# Autodesk Inventor assembly: ASY МОО 001 отстойник осветлитель
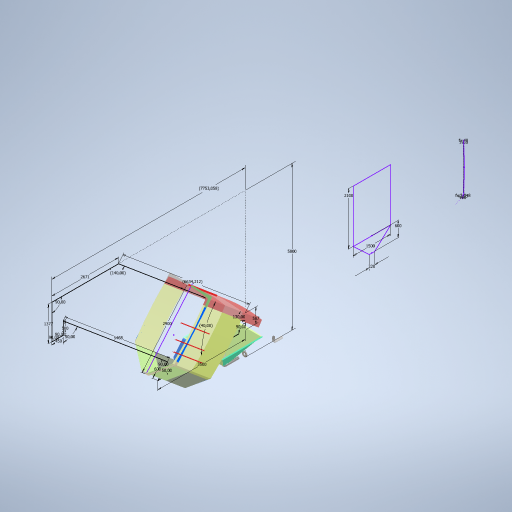
[picture p0: Inventor's stored thumbnail of the model, 512x512]
Saved by Autodesk Inventor 2024.2 (Build 282272000, 272)
## iProperties
Created: 2024-04-28
Part Number: ASY МОО 001 отстойник осветлитель
Document SubType Name: Weldment
Designer: admin
Weld Material: Welded Aluminum-6061
Mass: 420020 g
Surface Area: 719213 cm^2
Volume: 106788 cm^3
Density: 3.93322 g/cm^3
Author: admin
## Documents named in this file (23)
- C:\Users\user\YandexDisk\домашниий пк\Inventor\Manturovo\Manturovo_Se-clar\ASY МОО 001 отстойник осветлитель.iam
- C:\Users\user\YandexDisk\домашниий пк\Inventor\Manturovo\Manturovo_Se-clar\МОО 020 лист борт 1.ipt
- C:\Users\user\YandexDisk\домашниий пк\Inventor\Manturovo\Manturovo_Se-clar\МОО 010 лист спина 1.ipt
- C:\Users\user\YandexDisk\домашниий пк\Inventor\Manturovo\Manturovo_Se-clar\Пример емкости.ipt
- C:\Users\user\YandexDisk\домашниий пк\Inventor\Manturovo\Manturovo_Se-clar\МОО 030 лист брюхо 1.ipt
- C:\Users\user\YandexDisk\домашниий пк\Inventor\Manturovo\Manturovo_Se-clar\МОО 040 шпангоут борт 1.ipt
- C:\Users\user\YandexDisk\домашниий пк\Inventor\Manturovo\Manturovo_Se-clar\МОО 041 шпангоут спина 1.ipt
- C:\Users\user\YandexDisk\домашниий пк\Inventor\Manturovo\Manturovo_Se-clar\МОО 050 стрингер спина 1.ipt
- C:\Users\user\YandexDisk\домашниий пк\Inventor\Manturovo\Manturovo_Se-clar\Рама основания\ASY МОО 040 рама основания.iam
- C:\Users\user\YandexDisk\домашниий пк\Inventor\Manturovo\Manturovo_Se-clar\ASY МОО 060 ракета.iam
- C:\Users\user\YandexDisk\домашниий пк\Inventor\Manturovo\Manturovo_Se-clar\Content Center Files\en-US\ISO 5251 B 3D\ISO 5251 Bends 3D without straight ends(90 deg) DN80 2 2.ipt
- C:\Users\user\YandexDisk\домашниий пк\Inventor\Manturovo\Manturovo_Se-clar\Content Center Files\en-US\ISO 5251(1)\ISO 5251 Concentric reducers DN80 x DN65 3,2 3,2.ipt
- C:\Users\user\YandexDisk\домашниий пк\Inventor\Manturovo\Manturovo_Se-clar\ASY МОО 020 конус.iam
- C:\Users\user\YandexDisk\домашниий пк\Inventor\Manturovo\Manturovo_Se-clar\ракета\МОО 064 ракета труба.ipt
- C:\Users\user\YandexDisk\домашниий пк\Inventor\Manturovo\Manturovo_Se-clar\х_размеры МОО отстойник осветлитель Dummu.ipt
- C:\Users\user\YandexDisk\домашниий пк\Inventor\Manturovo\Manturovo_Se-clar\МОО 012 лист спина 2.ipt
- C:\Users\user\YandexDisk\домашниий пк\Inventor\Manturovo\Manturovo_Se-clar\ракета\МОО 065 ракета труба 5.ipt
- C:\Users\user\YandexDisk\домашниий пк\Inventor\Manturovo\Manturovo_Se-clar\ракета\МОО 066 ракета труба 6.ipt
- C:\Users\user\YandexDisk\домашниий пк\Inventor\Manturovo\Manturovo_Se-clar\ракета\МОО 067 ракета труба 7.ipt
- C:\Users\user\YandexDisk\домашниий пк\Inventor\Manturovo\Manturovo_Se-clar\Content Center Files\en-US\DIN EN 1092-1 01 - PN 25\DIN EN 1092-1 Plate Flange for Welding Type 01 - PN 25 80 x 88.9.ipt
- C:\Users\user\YandexDisk\домашниий пк\Inventor\Manturovo\Manturovo_Se-clar\МОО 011 лист борт.ipt
- C:\Users\user\YandexDisk\домашниий пк\Inventor\Manturovo\Manturovo_Se-clar\Листы бака Глеб\МОО 031 Усилитель спина.ipt
- C:\Users\user\YandexDisk\домашниий пк\Inventor\Manturovo\Manturovo_Se-clar\Листы бака Глеб\032 Усилитель левый борт.ipt
## Components (37 placed, 22 different names)
1. Пример емкости:1 — Mate:1, Mate:2, Flush:2
2. х_размеры МОО отстойник осветлитель Dummu:1
3. ASY МОО 040 рама основания:1 [sub-assembly] — Flush:19, Flush:20, Flush:21
4. МОО 020 лист борт 1:2 — Angle:1
5. МОО 010 лист спина 1:1 — Flush:3, Rigid:11, Rigid:12
6. МОО 020 лист борт 1:1 — Rigid:21, Rigid:22
7. МОО 030 лист брюхо 1:1 — Mate:9, Flush:29, Mate:21, Rigid:18
8. МОО 040 шпангоут борт 1:2 — Rigid:20
9. МОО 041 шпангоут спина 1:2 — Flush:12, Flush:33, Tangent:3, Rigid:15, Rigid:19, Flush:37
10. МОО 040 шпангоут борт 1:1 — Rigid:15, Flush:34, Rigid:21, Mate:23, Flush:35, Mate:24, Flush:36
11. МОО 050 стрингер спина 1:2 — Flush:34, Mate:23
12. ASY МОО 060 ракета:1 [sub-assembly] — Flush:23, Rigid:10
13. ISO 5251 Bends 3D without straight ends(90 deg) DN80 2:1 — Rigid:2, Rigid:3
14. ISO 5251 Concentric reducers DN80 x DN65 3,2:1 — Rigid:2, Rigid:10
15. ASY МОО 020 конус:1 [sub-assembly] — Flush:22, Mate:16, Flush:28
16. МОО 064 ракета труба:1 — Rigid:3, Cylindrical:1
17. МОО 010 лист спина 1:2 — Rigid:11, Rigid:13, Flush:31, Tangent:1, Flush:32, Tangent:2, Flush:33, Tangent:3
18. МОО 010 лист спина 1:3 — Flush:24, Rigid:12, Mate:19, Mate:22
19. МОО 012 лист спина 2:1 — Mate:15, Mate:16, Flush:27, Mate:19, Mate:22
20. МОО 065 ракета труба 5:1 — Rigid:5
21. МОО 066 ракета труба 6:1 — Rigid:5, Rigid:6
22. МОО 067 ракета труба 7:1 — Rigid:6, Rigid:7
23. DIN EN 1092-1 Plate Flange for Welding Type 01 - PN 25 80 x 88.9:1 — Flush:25, Flush:26, Mate:18, Cylindrical:1
24. ISO 5251 Concentric reducers DN80 x DN65 3,2:2 — Rigid:7
25. МОО 010 лист спина 1:4 — Rigid:13
26. МОО 011 лист борт:1 — Flush:30, Flush:31, Tangent:1, Rigid:16
27. МОО 011 лист борт:2 — Flush:29, Mate:20, Flush:32, Tangent:2, Mate:21
28. МОО 031 Усилитель спина:1
29. 032 Усилитель левый борт:1
30. МОО 041 шпангоут спина 1:3 — Rigid:19, Rigid:20
31. МОО 011 лист борт:3 — Rigid:16, Rigid:17
32. МОО 011 лист борт:4 — Rigid:17
33. МОО 030 лист брюхо 1:2 — Rigid:18
34. МОО 020 лист борт 1:3 — Rigid:22
35. МОО 050 стрингер спина 1:3 — Flush:35, Mate:24
36. МОО 050 стрингер спина 1:4 — Flush:36
37. МОО 050 стрингер спина 1:5 — Flush:37
## Relationships (56: Flush 22, WeldJoint 17, Mate 12, Tangent 3, Angle 1, CylindricalJoint 1)
- Mate:1: Пример емкости:1
- Mate:2: Пример емкости:1
- Flush:2: Пример емкости:1
- Flush:3: МОО 010 лист спина 1:1
- Angle:1 (180 deg): МОО 020 лист борт 1:2
- Mate:9: МОО 030 лист брюхо 1:1
- Flush:12: МОО 041 шпангоут спина 1:2
- Rigid:2 [WeldJoint]: ISO 5251 Bends 3D without straight ends(90 deg) DN80 2:1 ↔ ISO 5251 Concentric reducers DN80 x DN65 3,2:1
- Rigid:3 [WeldJoint]: ISO 5251 Bends 3D without straight ends(90 deg) DN80 2:1 ↔ МОО 064 ракета труба:1
- Flush:19 (-250 mm): ASY МОО 040 рама основания:1
- Flush:20: ASY МОО 040 рама основания:1
- Flush:21: ASY МОО 040 рама основания:1
- Flush:22: ASY МОО 020 конус:1
- Flush:23: ASY МОО 060 ракета:1
- Mate:15: МОО 012 лист спина 2:1
- Flush:24: МОО 010 лист спина 1:3
- Mate:16: ASY МОО 020 конус:1 ↔ МОО 012 лист спина 2:1
- Rigid:5 [WeldJoint]: МОО 065 ракета труба 5:1 ↔ МОО 066 ракета труба 6:1
- Rigid:6 [WeldJoint]: МОО 066 ракета труба 6:1 ↔ МОО 067 ракета труба 7:1
- Flush:25: DIN EN 1092-1 Plate Flange for Welding Type 01 - PN 25 80 x 88.9:1
- Flush:26: DIN EN 1092-1 Plate Flange for Welding Type 01 - PN 25 80 x 88.9:1
- Mate:18 (120 mm): DIN EN 1092-1 Plate Flange for Welding Type 01 - PN 25 80 x 88.9:1
- Rigid:7 [WeldJoint]: МОО 067 ракета труба 7:1 ↔ ISO 5251 Concentric reducers DN80 x DN65 3,2:2
- Rigid:10 [WeldJoint] (-20 mm): ASY МОО 060 ракета:1 ↔ ISO 5251 Concentric reducers DN80 x DN65 3,2:1
- Cylindrical:1: МОО 064 ракета труба:1 ↔ DIN EN 1092-1 Plate Flange for Welding Type 01 - PN 25 80 x 88.9:1
- Flush:27 (40 mm): МОО 012 лист спина 2:1
- Flush:28: ASY МОО 020 конус:1
- Rigid:11 [WeldJoint]: МОО 010 лист спина 1:1 ↔ МОО 010 лист спина 1:2
- Rigid:12 [WeldJoint] (-70 mm): МОО 010 лист спина 1:1 ↔ МОО 010 лист спина 1:3
- Mate:19: МОО 010 лист спина 1:3 ↔ МОО 012 лист спина 2:1
- Rigid:13 [WeldJoint]: МОО 010 лист спина 1:2 ↔ МОО 010 лист спина 1:4
- Flush:29: МОО 030 лист брюхо 1:1 ↔ МОО 011 лист борт:2
- Flush:30: МОО 011 лист борт:1
- Flush:31: МОО 010 лист спина 1:2 ↔ МОО 011 лист борт:1
- Tangent:1: МОО 010 лист спина 1:2 ↔ МОО 011 лист борт:1
- Mate:20: МОО 011 лист борт:2
- Flush:32: МОО 010 лист спина 1:2 ↔ МОО 011 лист борт:2
- Tangent:2: МОО 010 лист спина 1:2 ↔ МОО 011 лист борт:2
- Mate:21: МОО 030 лист брюхо 1:1 ↔ МОО 011 лист борт:2
- Flush:33 (100 mm): МОО 041 шпангоут спина 1:2 ↔ МОО 010 лист спина 1:2
- Tangent:3: МОО 041 шпангоут спина 1:2 ↔ МОО 010 лист спина 1:2
- Rigid:15 [WeldJoint]: МОО 041 шпангоут спина 1:2 ↔ МОО 040 шпангоут борт 1:1
- Mate:22 (47 mm): МОО 010 лист спина 1:3 ↔ МОО 012 лист спина 2:1
- Rigid:16 [WeldJoint]: МОО 011 лист борт:1 ↔ МОО 011 лист борт:3
- Rigid:17 [WeldJoint]: МОО 011 лист борт:3 ↔ МОО 011 лист борт:4
- Rigid:18 [WeldJoint]: МОО 030 лист брюхо 1:1 ↔ МОО 030 лист брюхо 1:2
- Rigid:19 [WeldJoint]: МОО 041 шпангоут спина 1:2 ↔ МОО 041 шпангоут спина 1:3
- Flush:34: МОО 040 шпангоут борт 1:1 ↔ МОО 050 стрингер спина 1:2
- Rigid:20 [WeldJoint]: МОО 040 шпангоут борт 1:2 ↔ МОО 041 шпангоут спина 1:3
- Rigid:21 [WeldJoint]: МОО 020 лист борт 1:1 ↔ МОО 040 шпангоут борт 1:1
- Rigid:22 [WeldJoint]: МОО 020 лист борт 1:1 ↔ МОО 020 лист борт 1:3
- Mate:23 (0.1 mm): МОО 040 шпангоут борт 1:1 ↔ МОО 050 стрингер спина 1:2
- Flush:35: МОО 040 шпангоут борт 1:1 ↔ МОО 050 стрингер спина 1:3
- Mate:24: МОО 040 шпангоут борт 1:1 ↔ МОО 050 стрингер спина 1:3
- Flush:36: МОО 040 шпангоут борт 1:1 ↔ МОО 050 стрингер спина 1:4
- Flush:37: МОО 041 шпангоут спина 1:2 ↔ МОО 050 стрингер спина 1:5
## Named parameters: Бак_нахлест_фланца = 25 mm
